# Autodesk Inventor assembly: 000-hand-grab-v2
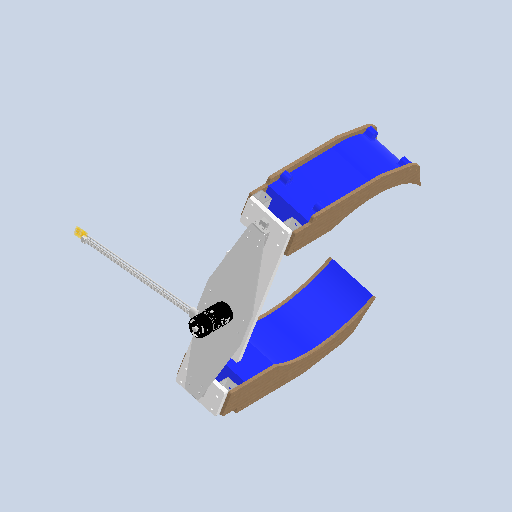
[picture p0: Inventor's stored thumbnail of the model, 512x512]
Saved by Autodesk Inventor 2025.1 (Build 291241000, 241)
## iProperties
Created: 2024-10-12
Part Number: 000-hand-grab-v2
Document SubType Name: Assembly
Designer: haruy
Author: haruy
## Documents named in this file (11)
- C:\Users\haruy\Documents\ロボコン\NHK2025\cad\nagahisa\hand\grab\000-hand-grab-v2.iam
- C:\Users\haruy\Documents\ロボコン\NHK2025\cad\nagahisa\hand\grab\hand-grab-v1-Plate-arm.ipt
- C:\Users\haruy\Documents\ロボコン\NHK2025\cad\nagahisa\hand\grab\hand-grab-v2-Plate-rack.ipt
- C:\Users\haruy\Documents\ロボコン\NHK2025\cad\nagahisa\hand\grab\SSEBZ-MX10-95.iam
- C:\Users\haruy\Documents\ロボコン\NHK2025\cad\nagahisa\hand\grab\hand-grab-v2-Plate-m=F.ipt
- C:\Users\haruy\Documents\ロボコン\NHK2025\cad\000_parts\モーター\robomaster\M2006 P36\RoboMaster M2006 P36\RoboMaster M2006 P36.ipt
- C:\Users\haruy\Documents\ロボコン\NHK2025\cad\nagahisa\hand\grab\000-hand-grab-v2\デザイン アクセラレータ\平歯車1.iam
- C:\Users\haruy\Documents\ロボコン\NHK2025\cad\nagahisa\hand\roller\SCSWJ6-6_b.ipt
- C:\Users\haruy\Documents\ロボコン\NHK2025\cad\nagahisa\hand\grab\hand-grab-v2-3DP-arm-C.ipt
- C:\Users\haruy\Documents\ロボコン\NHK2025\cad\nagahisa\hand\grab\hand-grab-v2-ASP-arm-F-1.ipt
- C:\Users\haruy\Documents\ロボコン\NHK2025\cad\nagahisa\hand\grab\hand-grab-v2-ASP-arm-support.ipt
## Components (20 placed, 10 different names)
1. hand-grab-v1-Plate-arm:1 — 挿入:32, 挿入:33, 挿入:46, 挿入:47
2. hand-grab-v2-Plate-rack:1 — 挿入:5, 挿入:6, 挿入:28, 挿入:29, 挿入:30, 挿入:31
3. hand-grab-v1-Plate-arm:2 — 挿入:44, 挿入:45
4. SSEBZ-MX10-95:1 [sub-assembly] — 挿入:5, 挿入:6, 挿入:7, 挿入:8
5. hand-grab-v2-Plate-m=F:1 — 挿入:7, 挿入:8, 挿入:15, 挿入:16, 挿入:17, 挿入:26, 挿入:48, 挿入:49, 挿入:50, 挿入:51
6. hand-grab-v1-Plate-arm:3 — 挿入:38, 挿入:39, 挿入:40, 挿入:41
7. hand-grab-v2-Plate-rack:2 — 挿入:34, 挿入:35, 挿入:36, 挿入:37
8. hand-grab-v1-Plate-arm:4 — 挿入:42, 挿入:43
9. SSEBZ-MX10-95:2 [sub-assembly] — 挿入:15, 挿入:16
10. RoboMaster M2006 P36:1 — 挿入:17, メイト:1
11. 平歯車:1 [sub-assembly] — 挿入:27, メイト:1
12. SCSWJ6-6_b:1 — 挿入:26, 挿入:27
13. hand-grab-v2-3DP-arm-C:1 — 挿入:44, 挿入:45, 挿入:46, 挿入:47
14. hand-grab-v2-3DP-arm-C:2 — 挿入:40, 挿入:41, 挿入:42, 挿入:43
15. hand-grab-v2-ASP-arm-F-1:1 — 挿入:30, 挿入:31
16. hand-grab-v2-ASP-arm-F-1:2 — 挿入:28, 挿入:29, 挿入:32, 挿入:33
17. hand-grab-v2-ASP-arm-F-1:3 — 挿入:34, 挿入:35
18. hand-grab-v2-ASP-arm-F-1:4 — 挿入:36, 挿入:37, 挿入:38, 挿入:39
19. hand-grab-v2-ASP-arm-support:1 — 挿入:48, 挿入:49
20. hand-grab-v2-ASP-arm-support:2 — 挿入:50, 挿入:51
## Relationships (36: Insert 35, Mate 1)
- 挿入:5 [Insert]: hand-grab-v2-Plate-rack:1 ↔ SSEBZ-MX10-95:1
- 挿入:6 [Insert]: hand-grab-v2-Plate-rack:1 ↔ SSEBZ-MX10-95:1
- 挿入:7 [Insert]: SSEBZ-MX10-95:1 ↔ hand-grab-v2-Plate-m=F:1
- 挿入:8 [Insert]: SSEBZ-MX10-95:1 ↔ hand-grab-v2-Plate-m=F:1
- [Insert]: hand-grab-v2-Plate-rack:2 ↔ SSEBZ-MX10-95:2
- [Insert]: hand-grab-v2-Plate-rack:2 ↔ SSEBZ-MX10-95:2
- 挿入:15 [Insert]: hand-grab-v2-Plate-m=F:1 ↔ SSEBZ-MX10-95:2
- 挿入:16 [Insert]: hand-grab-v2-Plate-m=F:1 ↔ SSEBZ-MX10-95:2
- 挿入:17 [Insert]: hand-grab-v2-Plate-m=F:1 ↔ RoboMaster M2006 P36:1
- 挿入:26 [Insert] (4 mm): hand-grab-v2-Plate-m=F:1 ↔ SCSWJ6-6_b:1
- 挿入:27 [Insert]: 平歯車:1 ↔ SCSWJ6-6_b:1
- 挿入:28 [Insert]: hand-grab-v2-Plate-rack:1 ↔ hand-grab-v2-ASP-arm-F-1:2
- 挿入:29 [Insert]: hand-grab-v2-Plate-rack:1 ↔ hand-grab-v2-ASP-arm-F-1:2
- 挿入:30 [Insert]: hand-grab-v2-Plate-rack:1 ↔ hand-grab-v2-ASP-arm-F-1:1
- 挿入:31 [Insert]: hand-grab-v2-Plate-rack:1 ↔ hand-grab-v2-ASP-arm-F-1:1
- 挿入:32 [Insert]: hand-grab-v1-Plate-arm:1 ↔ hand-grab-v2-ASP-arm-F-1:2
- 挿入:33 [Insert]: hand-grab-v1-Plate-arm:1 ↔ hand-grab-v2-ASP-arm-F-1:2
- 挿入:34 [Insert]: hand-grab-v2-Plate-rack:2 ↔ hand-grab-v2-ASP-arm-F-1:3
- 挿入:35 [Insert]: hand-grab-v2-Plate-rack:2 ↔ hand-grab-v2-ASP-arm-F-1:3
- 挿入:36 [Insert]: hand-grab-v2-Plate-rack:2 ↔ hand-grab-v2-ASP-arm-F-1:4
- 挿入:37 [Insert]: hand-grab-v2-Plate-rack:2 ↔ hand-grab-v2-ASP-arm-F-1:4
- 挿入:38 [Insert]: hand-grab-v1-Plate-arm:3 ↔ hand-grab-v2-ASP-arm-F-1:4
- 挿入:39 [Insert]: hand-grab-v1-Plate-arm:3 ↔ hand-grab-v2-ASP-arm-F-1:4
- 挿入:40 [Insert]: hand-grab-v1-Plate-arm:3 ↔ hand-grab-v2-3DP-arm-C:2
- 挿入:41 [Insert]: hand-grab-v1-Plate-arm:3 ↔ hand-grab-v2-3DP-arm-C:2
- 挿入:42 [Insert]: hand-grab-v1-Plate-arm:4 ↔ hand-grab-v2-3DP-arm-C:2
- 挿入:43 [Insert]: hand-grab-v1-Plate-arm:4 ↔ hand-grab-v2-3DP-arm-C:2
- 挿入:44 [Insert]: hand-grab-v1-Plate-arm:2 ↔ hand-grab-v2-3DP-arm-C:1
- 挿入:45 [Insert]: hand-grab-v1-Plate-arm:2 ↔ hand-grab-v2-3DP-arm-C:1
- 挿入:46 [Insert]: hand-grab-v1-Plate-arm:1 ↔ hand-grab-v2-3DP-arm-C:1
- 挿入:47 [Insert]: hand-grab-v1-Plate-arm:1 ↔ hand-grab-v2-3DP-arm-C:1
- 挿入:48 [Insert]: hand-grab-v2-Plate-m=F:1 ↔ hand-grab-v2-ASP-arm-support:1
- 挿入:49 [Insert]: hand-grab-v2-Plate-m=F:1 ↔ hand-grab-v2-ASP-arm-support:1
- 挿入:50 [Insert]: hand-grab-v2-Plate-m=F:1 ↔ hand-grab-v2-ASP-arm-support:2
- 挿入:51 [Insert]: hand-grab-v2-Plate-m=F:1 ↔ hand-grab-v2-ASP-arm-support:2
- メイト:1 [Mate]: RoboMaster M2006 P36:1 ↔ 平歯車:1
## Named parameters: d12_d4 = 0 mm, d13_d5 = 0 mm
